# Autodesk Inventor assembly: 4_Mecanum_Wheel_276-1447
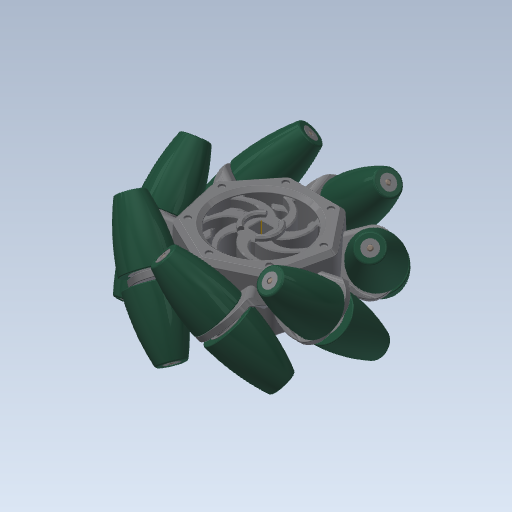
[picture p0: Inventor's stored thumbnail of the model, 512x512]
Saved by Autodesk Inventor 2020 (Build 240168000, 168)
## iProperties
Created: 2018-08-22
Part Number: 4_Mecanum_Wheel_276-1447
Material: 常规
Description: STEP AP214
Document SubType Name: Assembly
Designer: aresp
Sending System: SolidWorks 2017
Preprocessor: SwSTEP 2.0
Title: 217-1477-000 Rev3.STEP
Revision Number: ANY
## Documents named in this file (4)
- D:\vault\ncrCadLib\轮子\万向轮右前左后.iam
- D:\vault\ncrCadLib\轮子\Components\276-1447-002 Rev3.ipt
- D:\vault\ncrCadLib\轮子\Components\276-1447-001 Rev3.ipt
- D:\vault\ncrCadLib\轮子\Components\276-1447-010 Rev1.iam
## Components (9 placed, 9 different names)
1. 276-1447-002 Rev3_1 — 配合:1
2. 276-1447-001 Rev3_2 — 配合:2
3. 276-1447-010 Rev1_3 [sub-assembly]
4. 276-1447-010 Rev1_4 [sub-assembly]
5. 276-1447-010 Rev1_5 [sub-assembly]
6. 276-1447-010 Rev1_6 [sub-assembly]
7. 276-1447-010 Rev1_7 [sub-assembly]
8. 276-1447-010 Rev1_8 [sub-assembly]
9. 276-1447-010 Rev1_9 [sub-assembly]
## Relationships (2: Mate 2)
- 配合:1 [Mate]: 276-1447-002 Rev3_1
- 配合:2 [Mate]: 276-1447-001 Rev3_2
